# Autodesk Inventor assembly: SwerveDrive Model V2
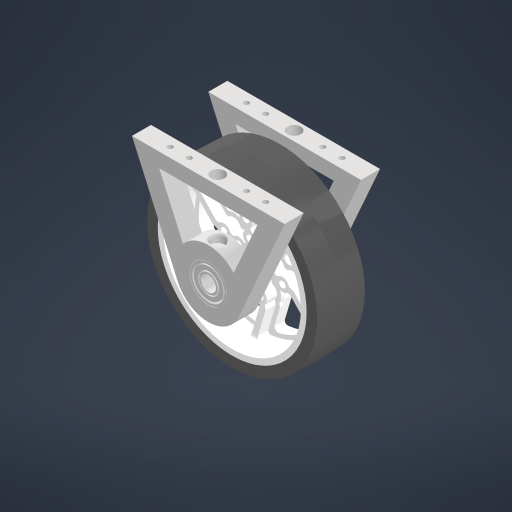
[picture p0: Inventor's stored thumbnail of the model, 512x512]
Saved by Autodesk Inventor 2023 (Build 270158000, 158)
## iProperties
Created: 2023-02-25
Part Number: SwerveDrive Model V2
Document SubType Name: Assembly
Designer: izack
Author: izack
## Documents named in this file (5)
- D:\Robotics\Custom-Modules-CAD\SwerveDrive V2\SwerveDrive Model V2.iam
- D:\Robotics\Custom-Modules-CAD\SwerveDrive V2\SwerveDrive V2 Parts\90mm Grip Wheel.iam
- 90mm Grip Wheel.iam
- D:\Robotics\Custom-Modules-CAD\SwerveDrive V2\SwerveDrive V2 Parts\LowerWheelBracket.ipt
- D:\Robotics\Custom-Modules-CAD\Bearings V2\Bearing V2.iam
## Components (7 placed, 3 different names)
1. 90mm Grip Wheel:1 [sub-assembly] — Flush:1, Flush:2, Mate:4
2. LowerWheelBracket:1 — Flush:1, Flush:2, Mate:1, Flush:3, Mate:3, Flush:5, Mate:4, Mate:5, Flush:6
3. 19.5mm_Bearing V2:1 [sub-assembly] — Mate:1, Flush:3, Mate:2
4. 19.5mm_Bearing V2:2 [sub-assembly] — Mate:2, Mate:3
5. 19.5mm_Bearing V2:3 [sub-assembly] — Mate:7, Mate:8
6. 19.5mm_Bearing V2:4 [sub-assembly] — Mate:6, Flush:7, Mate:7
7. LowerWheelBracket:2 — Flush:5, Mate:5, Flush:6, Mate:6, Flush:7, Mate:8
## Relationships (14: Mate 8, Flush 6)
- Flush:1: 90mm Grip Wheel:1 ↔ LowerWheelBracket:1
- Flush:2 (2.5 mm): 90mm Grip Wheel:1 ↔ LowerWheelBracket:1
- Mate:1: LowerWheelBracket:1 ↔ 19.5mm_Bearing V2:1
- Flush:3: LowerWheelBracket:1 ↔ 19.5mm_Bearing V2:1
- Mate:2: 19.5mm_Bearing V2:1 ↔ 19.5mm_Bearing V2:2
- Mate:3: LowerWheelBracket:1 ↔ 19.5mm_Bearing V2:2
- Flush:5: LowerWheelBracket:1 ↔ LowerWheelBracket:2
- Mate:4: 90mm Grip Wheel:1 ↔ LowerWheelBracket:1
- Mate:5 (30 mm): LowerWheelBracket:1 ↔ LowerWheelBracket:2
- Flush:6: LowerWheelBracket:1 ↔ LowerWheelBracket:2
- Mate:6: 19.5mm_Bearing V2:4 ↔ LowerWheelBracket:2
- Flush:7: 19.5mm_Bearing V2:4 ↔ LowerWheelBracket:2
- Mate:7: 19.5mm_Bearing V2:3 ↔ 19.5mm_Bearing V2:4
- Mate:8: 19.5mm_Bearing V2:3 ↔ LowerWheelBracket:2
